# Autodesk Inventor assembly: ElectronicsV2
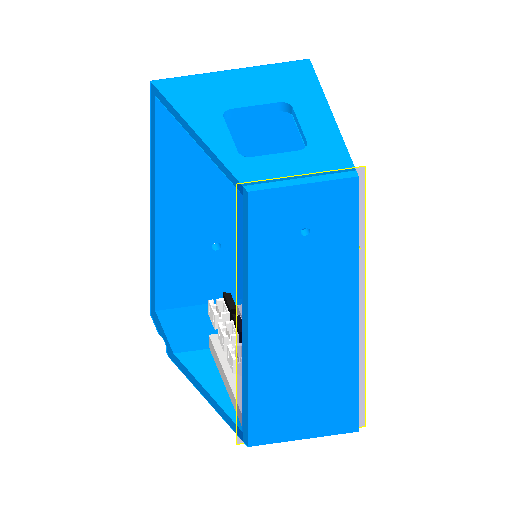
[picture p0: Inventor's stored thumbnail of the model, 512x512]
Saved by Autodesk Inventor 2025.1 (Build 291241020, 241B)
## iProperties
Created: 2025-08-04
Part Number: ElectronicsV2
Document SubType Name: Assembly
Designer: jaschreiner
Author: jaschreiner
## Documents named in this file (8)
- C:\Users\jaschreiner\Documents\FAPS\Forschung\ToCaro\CAD Dateien\ElectronicsV2.iam
- C:\Users\jaschreiner\Documents\FAPS\Forschung\ToCaro\CAD Dateien\Motorhalter Electronics Box V4.ipt
- C:\Users\jaschreiner\Documents\FAPS\Forschung\ToCaro\CAD Dateien\ruthex_RX-M3x4.0_SHORT\ruthex_RX-M3x4.0_SHORT\ruthex RX-M3-5,7.ipt
- C:\Users\jaschreiner\Documents\FAPS\Forschung\ToCaro\CAD Dateien\Gearmotor, Micro Metal, 50.1, with Driver\Gearmotor, Micro Metal, 50.1, with Driver\Gearmotor, Micro Metal, 50.1, with Driver.iam
- C:\Users\jaschreiner\Documents\FAPS\Forschung\ToCaro\CAD Dateien\Seilwinde.ipt
- C:\Users\jaschreiner\OneDrive - Friedrich-Alexander Universität Erlangen-Nürnberg\Dokumente\Inventor\Content Center Files\R2025\de-DE\ISO 10642(2)\ISO 10642  - M3  x  8.ipt
- C:\Users\jaschreiner\Documents\FAPS\Forschung\ToCaro\CAD Dateien\Electronics Box V5.ipt
- C:\Users\jaschreiner\Documents\FAPS\Forschung\Experiment!Material\Tube1.ipt
## Components (20 placed, 7 different names)
1. Motorhalter Electronics Box V4:1 — Passend:4, Passend:5, Passend:6, Passend:7, Passend:8, Passend:9, Passend:11, Passend:12, Passend:17, Starr:1, Starr:2, Starr:3, Starr:4
2. ruthex RX-M3-5,7:1 — Starr:1, Drehbar:10
3. ruthex RX-M3-5,7:2 — Starr:4
4. ruthex RX-M3-5,7:3 — Starr:3, Drehbar:11
5. ruthex RX-M3-5,7:4 — Starr:2
6. Gearmotor, Micro Metal, 50.1, with Driver:1 [sub-assembly] — Passend:11, Passend:12, Drehbar:7, Passend:17
7. Gearmotor, Micro Metal, 50.1, with Driver:2 [sub-assembly] — Passend:7, Passend:8, Passend:9, Drehbar:8
8. Gearmotor, Micro Metal, 50.1, with Driver:3 [sub-assembly] — Passend:4, Passend:5, Passend:6, Drehbar:12
9. Seilwinde:1 — Drehbar:12
10. Seilwinde:2 — Drehbar:8
11. Seilwinde:3 — Drehbar:7
12. DIN EN ISO 10642 M3  x  8:1 — Passend:18
13. DIN EN ISO 10642 M3  x  8:2 — Passend:19
14. DIN EN ISO 10642 M3  x  8:3 — Passend:20
15. DIN EN ISO 10642 M3  x  8:4 — Passend:21
16. Electronics Box V5:1 — Drehbar:10, Drehbar:11, Passend:18, Passend:19, Passend:20, Passend:21, Passend:22, Passend:23, Passend:24, Fluchtend:1, Fluchtend:2, Fluchtend:3
17. DIN EN ISO 10642 M3  x  8:5 — Passend:22
18. DIN EN ISO 10642 M3  x  8:6 — Passend:23
19. DIN EN ISO 10642 M3  x  8:7 — Passend:24
20. Tube1:1 — Fluchtend:1, Fluchtend:2, Fluchtend:3
## Relationships (28: Mate 16, RevoluteJoint 5, WeldJoint 4, Flush 3)
- Passend:4 [Mate]: Motorhalter Electronics Box V4:1 ↔ Gearmotor, Micro Metal, 50.1, with Driver:3
- Passend:5 [Mate] (0.05 mm): Motorhalter Electronics Box V4:1 ↔ Gearmotor, Micro Metal, 50.1, with Driver:3
- Passend:6 [Mate]: Motorhalter Electronics Box V4:1 ↔ Gearmotor, Micro Metal, 50.1, with Driver:3
- Passend:7 [Mate]: Motorhalter Electronics Box V4:1 ↔ Gearmotor, Micro Metal, 50.1, with Driver:2
- Passend:8 [Mate] (0.05 mm): Motorhalter Electronics Box V4:1 ↔ Gearmotor, Micro Metal, 50.1, with Driver:2
- Passend:9 [Mate]: Motorhalter Electronics Box V4:1 ↔ Gearmotor, Micro Metal, 50.1, with Driver:2
- Passend:11 [Mate] (0.05 mm): Motorhalter Electronics Box V4:1 ↔ Gearmotor, Micro Metal, 50.1, with Driver:1
- Passend:12 [Mate]: Motorhalter Electronics Box V4:1 ↔ Gearmotor, Micro Metal, 50.1, with Driver:1
- Drehbar:7 [RevoluteJoint]: Gearmotor, Micro Metal, 50.1, with Driver:1 ↔ Seilwinde:3
- Drehbar:8 [RevoluteJoint]: Gearmotor, Micro Metal, 50.1, with Driver:2 ↔ Seilwinde:2
- Passend:17 [Mate]: Motorhalter Electronics Box V4:1 ↔ Gearmotor, Micro Metal, 50.1, with Driver:1
- Starr:1 [WeldJoint]: Motorhalter Electronics Box V4:1 ↔ ruthex RX-M3-5,7:1
- Starr:2 [WeldJoint]: Motorhalter Electronics Box V4:1 ↔ ruthex RX-M3-5,7:4
- Starr:3 [WeldJoint]: Motorhalter Electronics Box V4:1 ↔ ruthex RX-M3-5,7:3
- Starr:4 [WeldJoint]: Motorhalter Electronics Box V4:1 ↔ ruthex RX-M3-5,7:2
- Drehbar:10 [RevoluteJoint]: ruthex RX-M3-5,7:1 ↔ Electronics Box V5:1
- Drehbar:11 [RevoluteJoint]: ruthex RX-M3-5,7:3 ↔ Electronics Box V5:1
- Passend:18 [Mate]: DIN EN ISO 10642 M3  x  8:1 ↔ Electronics Box V5:1
- Passend:19 [Mate]: DIN EN ISO 10642 M3  x  8:2 ↔ Electronics Box V5:1
- Passend:20 [Mate]: DIN EN ISO 10642 M3  x  8:3 ↔ Electronics Box V5:1
- Passend:21 [Mate]: DIN EN ISO 10642 M3  x  8:4 ↔ Electronics Box V5:1
- Passend:22 [Mate]: Electronics Box V5:1 ↔ DIN EN ISO 10642 M3  x  8:5
- Passend:23 [Mate]: Electronics Box V5:1 ↔ DIN EN ISO 10642 M3  x  8:6
- Passend:24 [Mate]: Electronics Box V5:1 ↔ DIN EN ISO 10642 M3  x  8:7
- Drehbar:12 [RevoluteJoint]: Gearmotor, Micro Metal, 50.1, with Driver:3 ↔ Seilwinde:1
- Fluchtend:1 [Flush]: Electronics Box V5:1 ↔ Tube1:1
- Fluchtend:2 [Flush]: Electronics Box V5:1 ↔ Tube1:1
- Fluchtend:3 [Flush]: Electronics Box V5:1 ↔ Tube1:1
